# Autodesk Inventor assembly: Full Roller Carousel Assembly
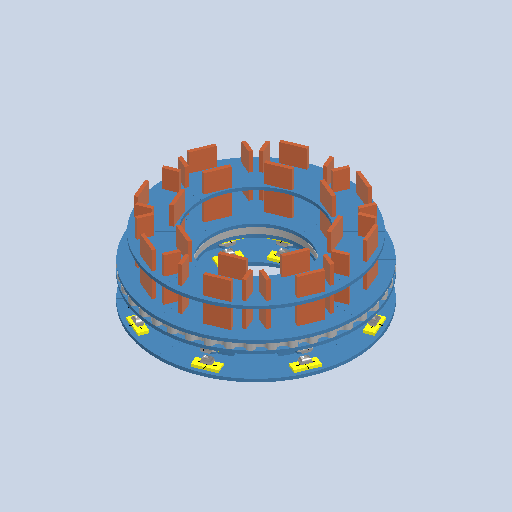
[picture p0: Inventor's stored thumbnail of the model, 512x512]
Saved by Autodesk Inventor 2023 (Build 270158000, 158)
## iProperties
Created: 2022-12-06
Part Number: Full Roller Carousel Assembly
Document SubType Name: Assembly
Designer: mihal
Author: mihal
## Documents named in this file (2)
- C:\Users\mihal\Desktop\Current BHSS Design\Eighth Assembly\Full Roller Carousel Assembly.iam
- C:\Users\mihal\Desktop\Current BHSS Design\Eighth Assembly\Roller Carouel Assembly.iam
## Components (8 placed, 1 different names)
1. Roller Carouel Assembly:1 [sub-assembly] — Mate:1, Mate:2, Mate:5
2. Roller Carouel Assembly:2 [sub-assembly] — Mate:1, Mate:2, Mate:3, Mate:4, Mate:5, Mate:6
3. Roller Carouel Assembly:3 [sub-assembly] — Mate:3, Mate:4, Mate:6, Mate:7, Mate:8, Mate:9
4. Roller Carouel Assembly:4 [sub-assembly] — Mate:7, Mate:8, Mate:9, Mate:10, Mate:11, Mate:12
5. Roller Carouel Assembly:5 [sub-assembly] — Mate:10, Mate:11, Mate:12, Mate:13, Mate:14, Mate:15
6. Roller Carouel Assembly:6 [sub-assembly] — Mate:13, Mate:14, Mate:15, Mate:16, Mate:17, Mate:18
7. Roller Carouel Assembly:7 [sub-assembly] — Mate:16, Mate:17, Mate:18, Mate:19, Mate:20, Mate:21
8. Roller Carouel Assembly:8 [sub-assembly] — Mate:19, Mate:20, Mate:21
## Relationships (21: Mate 21)
- Mate:1: Roller Carouel Assembly:1 ↔ Roller Carouel Assembly:2
- Mate:2: Roller Carouel Assembly:1 ↔ Roller Carouel Assembly:2
- Mate:3: Roller Carouel Assembly:2 ↔ Roller Carouel Assembly:3
- Mate:4: Roller Carouel Assembly:2 ↔ Roller Carouel Assembly:3
- Mate:5: Roller Carouel Assembly:1 ↔ Roller Carouel Assembly:2
- Mate:6: Roller Carouel Assembly:2 ↔ Roller Carouel Assembly:3
- Mate:7: Roller Carouel Assembly:3 ↔ Roller Carouel Assembly:4
- Mate:8: Roller Carouel Assembly:3 ↔ Roller Carouel Assembly:4
- Mate:9: Roller Carouel Assembly:3 ↔ Roller Carouel Assembly:4
- Mate:10: Roller Carouel Assembly:4 ↔ Roller Carouel Assembly:5
- Mate:11: Roller Carouel Assembly:4 ↔ Roller Carouel Assembly:5
- Mate:12: Roller Carouel Assembly:4 ↔ Roller Carouel Assembly:5
- Mate:13: Roller Carouel Assembly:5 ↔ Roller Carouel Assembly:6
- Mate:14: Roller Carouel Assembly:5 ↔ Roller Carouel Assembly:6
- Mate:15: Roller Carouel Assembly:5 ↔ Roller Carouel Assembly:6
- Mate:16: Roller Carouel Assembly:6 ↔ Roller Carouel Assembly:7
- Mate:17: Roller Carouel Assembly:6 ↔ Roller Carouel Assembly:7
- Mate:18: Roller Carouel Assembly:6 ↔ Roller Carouel Assembly:7
- Mate:19: Roller Carouel Assembly:7 ↔ Roller Carouel Assembly:8
- Mate:20: Roller Carouel Assembly:7 ↔ Roller Carouel Assembly:8
- Mate:21: Roller Carouel Assembly:7 ↔ Roller Carouel Assembly:8
